# Autodesk Inventor assembly: Wall Assembly
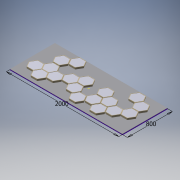
[picture p0: Inventor's stored thumbnail of the model, 180x180]
Saved by Autodesk Inventor 2019 (Build 230136000, 136)
## iProperties
Created: 2021-07-14
Part Number: Wall Assembly
Document SubType Name: Assembly
Designer: Lix
Author: Lix
## Documents named in this file (3)
- G:\Project\3d-printing\Models\My Own\Hexagonal Deco Lamp\Wall Assembly.iam
- G:\Project\3d-printing\Models\My Own\Hexagonal Deco Lamp\Wall.ipt
- G:\Project\3d-printing\Models\My Own\Hexagonal Deco Lamp\Hexagonal Deco Lamp Assembly.iam
## Components (19 placed, 2 different names)
1. Wall:1
2. Hexagonal Deco Lamp Assembly:1 [sub-assembly] — Flush:1, Flush:2, Flush:3, Flush:4, Mate:2, Mate:3
3. Hexagonal Deco Lamp Assembly:2 [sub-assembly] — Flush:1, Mate:1, Mate:2
4. Hexagonal Deco Lamp Assembly:3 [sub-assembly] — Flush:2, Mate:1, Mate:3
5. Hexagonal Deco Lamp Assembly:4 [sub-assembly] — Flush:3, Flush:6
6. Hexagonal Deco Lamp Assembly:5 [sub-assembly] — Flush:5
7. Hexagonal Deco Lamp Assembly:6 [sub-assembly] — Flush:4, Flush:5
8. Hexagonal Deco Lamp Assembly:7 [sub-assembly] — Flush:6, Flush:7, Flush:9
9. Hexagonal Deco Lamp Assembly:8 [sub-assembly] — Flush:7, Flush:8, Flush:9
10. Hexagonal Deco Lamp Assembly:9 [sub-assembly] — Flush:8, Flush:10
11. Hexagonal Deco Lamp Assembly:10 [sub-assembly] — Flush:11, Flush:12
12. Hexagonal Deco Lamp Assembly:11 [sub-assembly] — Flush:13, Flush:14, Flush:15
13. Hexagonal Deco Lamp Assembly:12 [sub-assembly] — Flush:15, Flush:16
14. Hexagonal Deco Lamp Assembly:13 [sub-assembly] — Flush:14
15. Hexagonal Deco Lamp Assembly:14 [sub-assembly] — Flush:10, Flush:11
16. Hexagonal Deco Lamp Assembly:15 [sub-assembly] — Flush:12, Flush:13
17. Hexagonal Deco Lamp Assembly:16 [sub-assembly] — Flush:16, Flush:17, Flush:18
18. Hexagonal Deco Lamp Assembly:17 [sub-assembly] — Flush:17, Flush:18, Flush:19
19. Hexagonal Deco Lamp Assembly:18 [sub-assembly] — Flush:19
## Relationships (22: Flush 19, Mate 3)
- Flush:1: Hexagonal Deco Lamp Assembly:1 ↔ Hexagonal Deco Lamp Assembly:2
- Flush:2: Hexagonal Deco Lamp Assembly:1 ↔ Hexagonal Deco Lamp Assembly:3
- Flush:3: Hexagonal Deco Lamp Assembly:1 ↔ Hexagonal Deco Lamp Assembly:4
- Flush:4: Hexagonal Deco Lamp Assembly:1 ↔ Hexagonal Deco Lamp Assembly:6
- Flush:5: Hexagonal Deco Lamp Assembly:5 ↔ Hexagonal Deco Lamp Assembly:6
- Flush:6: Hexagonal Deco Lamp Assembly:4 ↔ Hexagonal Deco Lamp Assembly:7
- Flush:7: Hexagonal Deco Lamp Assembly:7 ↔ Hexagonal Deco Lamp Assembly:8
- Flush:8: Hexagonal Deco Lamp Assembly:8 ↔ Hexagonal Deco Lamp Assembly:9
- Flush:9: Hexagonal Deco Lamp Assembly:7 ↔ Hexagonal Deco Lamp Assembly:8
- Flush:10: Hexagonal Deco Lamp Assembly:9 ↔ Hexagonal Deco Lamp Assembly:14
- Flush:11: Hexagonal Deco Lamp Assembly:10 ↔ Hexagonal Deco Lamp Assembly:14
- Flush:12: Hexagonal Deco Lamp Assembly:10 ↔ Hexagonal Deco Lamp Assembly:15
- Flush:13: Hexagonal Deco Lamp Assembly:11 ↔ Hexagonal Deco Lamp Assembly:15
- Flush:14: Hexagonal Deco Lamp Assembly:11 ↔ Hexagonal Deco Lamp Assembly:13
- Flush:15: Hexagonal Deco Lamp Assembly:11 ↔ Hexagonal Deco Lamp Assembly:12
- Flush:16: Hexagonal Deco Lamp Assembly:12 ↔ Hexagonal Deco Lamp Assembly:16
- Flush:17: Hexagonal Deco Lamp Assembly:16 ↔ Hexagonal Deco Lamp Assembly:17
- Flush:18: Hexagonal Deco Lamp Assembly:16 ↔ Hexagonal Deco Lamp Assembly:17
- Flush:19: Hexagonal Deco Lamp Assembly:17 ↔ Hexagonal Deco Lamp Assembly:18
- Mate:1: Hexagonal Deco Lamp Assembly:2 ↔ Hexagonal Deco Lamp Assembly:3
- Mate:2: Hexagonal Deco Lamp Assembly:1 ↔ Hexagonal Deco Lamp Assembly:2
- Mate:3: Hexagonal Deco Lamp Assembly:1 ↔ Hexagonal Deco Lamp Assembly:3
